# Autodesk Inventor assembly: KB33-046-002 - Рама
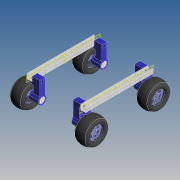
[picture p0: Inventor's stored thumbnail of the model, 180x180]
Saved by Autodesk Inventor 2020 (Build 240168000, 168)
## iProperties
Created: 2021-06-09
Part Number: KB33-046-002 - Рама
Material: Типовые
Document SubType Name: Assembly
Designer: Петров Иван
Mass: 5235.61 g
Surface Area: 8118.47 cm^2
Volume: 5115.5 cm^3
Density: 1.02348 g/cm^3
Author: Петров Иван
## Documents named in this file (4)
- E:\IVAN\Ivan_desktop\Kvantorium\Projects\RoboPatrol\design\KB33-046-001 - Ходовая часть.iam
- E:\IVAN\Ivan_desktop\Kvantorium\Projects\RoboPatrol\design\standart_components\Tetrix\ftc-tetrix-kit-of-parts-1.snapshot.34\MAX Channels\416mm Channel.ipt
- E:\IVAN\Ivan_desktop\Kvantorium\Projects\RoboPatrol\design\KB33-046-002 - Привод в сборе.iam
- E:\IVAN\Ivan_desktop\Kvantorium\Projects\RoboPatrol\design\KB33-046-003 - Рама центральная.iam
## Components (7 placed, 3 different names)
1. 416mm Channel:1 — Заподлицо:2, Заподлицо:3, Совмещение:1, Совмещение:4, Совмещение:6, Совмещение:8, Совмещение:9, Совмещение:10
2. 416mm Channel:2 — Заподлицо:1, Заподлицо:3, Совмещение:1, Угол:1, Заподлицо:4, Заподлицо:5, Заподлицо:6, Совмещение:2, Совмещение:3
3. KB33-046-002 - Привод в сборе:1 [sub-assembly] — Угол:1, Заподлицо:4, Заподлицо:5, Заподлицо:6
4. KB33-046-002 - Привод в сборе:2 [sub-assembly] — Совмещение:2, Совмещение:3
5. KB33-046-002 - Привод в сборе:3 [sub-assembly] — Совмещение:4, Совмещение:6, Совмещение:9
6. KB33-046-002 - Привод в сборе:4 [sub-assembly] — Совмещение:8, Совмещение:10
7. KB33-046-003 - Рама центральная:1 [sub-assembly]
## Relationships (15: Mate 8, Flush 6, Angle 1)
- Заподлицо:1 [Flush]: 416mm Channel:2
- Заподлицо:2 [Flush]: 416mm Channel:1
- Заподлицо:3 [Flush]: 416mm Channel:1 ↔ 416mm Channel:2
- Совмещение:1 [Mate] (300 mm): 416mm Channel:1 ↔ 416mm Channel:2
- Угол:1 [Angle] (0 deg): 416mm Channel:2 ↔ KB33-046-002 - Привод в сборе:1
- Заподлицо:4 [Flush] (15 mm): 416mm Channel:2 ↔ KB33-046-002 - Привод в сборе:1
- Заподлицо:5 [Flush]: 416mm Channel:2 ↔ KB33-046-002 - Привод в сборе:1
- Заподлицо:6 [Flush]: 416mm Channel:2 ↔ KB33-046-002 - Привод в сборе:1
- Совмещение:2 [Mate]: 416mm Channel:2 ↔ KB33-046-002 - Привод в сборе:2
- Совмещение:3 [Mate]: 416mm Channel:2 ↔ KB33-046-002 - Привод в сборе:2
- Совмещение:4 [Mate]: 416mm Channel:1 ↔ KB33-046-002 - Привод в сборе:3
- Совмещение:6 [Mate]: 416mm Channel:1 ↔ KB33-046-002 - Привод в сборе:3
- Совмещение:8 [Mate]: 416mm Channel:1 ↔ KB33-046-002 - Привод в сборе:4
- Совмещение:9 [Mate]: 416mm Channel:1 ↔ KB33-046-002 - Привод в сборе:3
- Совмещение:10 [Mate]: 416mm Channel:1 ↔ KB33-046-002 - Привод в сборе:4
